# Autodesk Inventor assembly: B_Drive
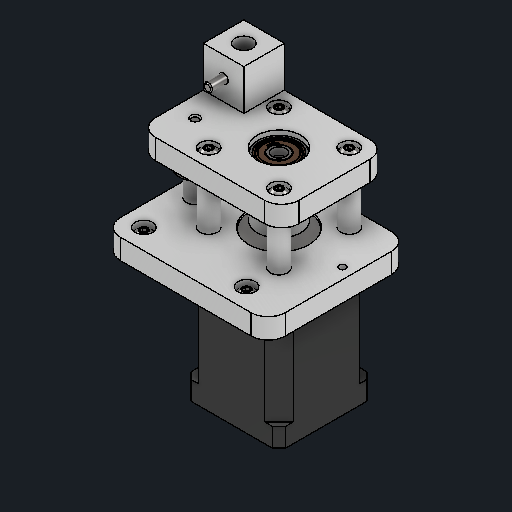
[picture p0: Inventor's stored thumbnail of the model, 512x512]
Saved by Autodesk Inventor 2026.1 (Build 301233020, 233B)
## iProperties
Created: 2025-05-24
Part Number: B_Drive
Document SubType Name: Assembly
Designer: Joshua Eah
Author: Joshua Eah
## Documents named in this file (14)
- C:\Users\JoshuaEah\Documents\GitHub\Voron-0\CAD\AB Drives\B Drive\B_Drive.iam
- C:\Users\JoshuaEah\Documents\GitHub\Voron-0\CAD\AB Drives\B Drive\B Drive Frame Lower.ipt
- C:\Users\JoshuaEah\Documents\GitHub\Voron-0\CAD\Spacers\Spacer.ipt
- C:\Users\JoshuaEah\Documents\GitHub\Voron-0\CAD\AB Drives\Drive Frame Spacer\Drive Frame Spacer.ipt
- C:\Users\JoshuaEah\Documents\GitHub\Voron-0\CAD\AB Drives\B Drive\B Drive Frame Upper.ipt
- C:\Users\JoshuaEah\Documents\GitHub\Voron-0\CAD\Hardware\3x30 Pin.ipt
- C:\Users\JoshuaEah\Documents\GitHub\Voron-0\CAD\Hardware\F623 Stack.iam
- C:\Users\JoshuaEah\Documents\GitHub\Voron-0\CAD\Hardware\M3x30 BHCS.ipt
- C:\Users\JoshuaEah\Documents\GitHub\Voron-0\CAD\Hardware\M3_Washer.ipt
- C:\Users\JoshuaEah\Documents\GitHub\Voron-0\CAD\Hardware\M3x10 BHCS.ipt
- C:\Users\JoshuaEah\Documents\GitHub\Voron-0\CAD\Electronics\Parts\Nema14.ipt
- C:\Users\JoshuaEah\Documents\GitHub\Voron-0\CAD\Hardware\GT2 20T 6mm Pulley.iam
- C:\Users\JoshuaEah\Documents\GitHub\Voron-0\CAD\Hardware\625ZZ Bearing.iam
- 625ZZ Bearing.iam
## Components (27 placed, 12 different names)
1. B Drive Frame Lower:1 — Insert:4, Insert:5, Insert:6, Insert:7, Insert:10, Insert:11, Insert:25, Insert:27, Insert:28, Insert:31, Insert:33, Insert:34, Insert:35
2. B Drive Frame Upper:1 — Insert:8, Insert:9, Mate:1, Mate:2, Insert:21, Insert:22, Insert:23, Insert:24, Insert:26, Insert:29
3. Spacer:1 — Insert:30, Insert:31
4. Drive Frame Spacer:3 — Insert:4
5. Drive Frame Spacer:4 — Insert:5, Insert:9
6. Drive Frame Spacer:5 — Insert:6
7. Drive Frame Spacer:6 — Insert:7, Insert:8
8. 3x30 Pin:1 — Mate:1, Insert:10
9. 3x30 Pin:2 — Mate:2, Insert:11
10. F623 Stack:1 [sub-assembly] — Insert:32
11. F623 Stack:2 [sub-assembly] — Insert:32, Insert:33
12. F623 Stack:3 [sub-assembly] — Insert:30
13. M3x30 BHCS:1 — Insert:17
14. M3x30 BHCS:2
15. M3x30 BHCS:3
16. M3x30 BHCS:4
17. M3_Washer:1 — Insert:17, Insert:21
18. M3_Washer:2 — Insert:22
19. M3_Washer:3 — Insert:23
20. M3_Washer:4 — Insert:24
21. M3x10 BHCS:1 — Insert:25
22. M3x10 BHCS:2 — Insert:26
23. M3x10 BHCS:3 — Insert:34
24. M3x10 BHCS:4 — Insert:35
25. Nema14:1 — Insert:27, Insert:28, Mate:3, Mate:4
26. GT2 20T 6mm Pulley:1 [sub-assembly] — Mate:3, Mate:4
27. 625ZZ Bearing:1 [sub-assembly] — Insert:29
## Relationships (31: Insert 27, Mate 4)
- Insert:4: B Drive Frame Lower:1 ↔ Drive Frame Spacer:3
- Insert:5: B Drive Frame Lower:1 ↔ Drive Frame Spacer:4
- Insert:6: B Drive Frame Lower:1 ↔ Drive Frame Spacer:5
- Insert:7: B Drive Frame Lower:1 ↔ Drive Frame Spacer:6
- Insert:8: B Drive Frame Upper:1 ↔ Drive Frame Spacer:6
- Insert:9: B Drive Frame Upper:1 ↔ Drive Frame Spacer:4
- Mate:1: B Drive Frame Upper:1 ↔ 3x30 Pin:1
- Mate:2: B Drive Frame Upper:1 ↔ 3x30 Pin:2
- Insert:10: B Drive Frame Lower:1 ↔ 3x30 Pin:1
- Insert:11: B Drive Frame Lower:1 ↔ 3x30 Pin:2
- Insert:17: M3x30 BHCS:1 ↔ M3_Washer:1
- [Insert]: M3x30 BHCS:2 ↔ M3_Washer:2
- [Insert]: M3x30 BHCS:3 ↔ M3_Washer:3
- [Insert]: M3x30 BHCS:4 ↔ M3_Washer:4
- Insert:21: B Drive Frame Upper:1 ↔ M3_Washer:1
- Insert:22: B Drive Frame Upper:1 ↔ M3_Washer:2
- Insert:23: B Drive Frame Upper:1 ↔ M3_Washer:3
- Insert:24: B Drive Frame Upper:1 ↔ M3_Washer:4
- Insert:25: B Drive Frame Lower:1 ↔ M3x10 BHCS:1
- Insert:26: B Drive Frame Upper:1 ↔ M3x10 BHCS:2
- Insert:27: B Drive Frame Lower:1 ↔ Nema14:1
- Insert:28: B Drive Frame Lower:1 ↔ Nema14:1
- Insert:29: B Drive Frame Upper:1 ↔ 625ZZ Bearing:1
- Mate:3: Nema14:1 ↔ GT2 20T 6mm Pulley:1
- Mate:4 (2.65 mm): Nema14:1 ↔ GT2 20T 6mm Pulley:1
- Insert:30: Spacer:1 ↔ F623 Stack:3
- Insert:31: B Drive Frame Lower:1 ↔ Spacer:1
- Insert:32: F623 Stack:1 ↔ F623 Stack:2
- Insert:33: B Drive Frame Lower:1 ↔ F623 Stack:2
- Insert:34: B Drive Frame Lower:1 ↔ M3x10 BHCS:3
- Insert:35: B Drive Frame Lower:1 ↔ M3x10 BHCS:4
## Named parameters: d19_d18 = 0 mm, d20_d18 = 0 mm, d21_d18 = 0 mm
